# Autodesk Inventor assembly: Cold Plate in Box
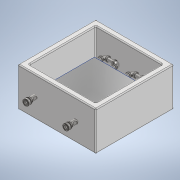
[picture p0: Inventor's stored thumbnail of the model, 180x180]
Saved by Autodesk Inventor 2022 (Build 260153000, 153)
## iProperties
Created: 2022-01-24
Part Number: Cold Plate in Box
Document SubType Name: Assembly
Designer: Caleb
Author: Caleb
## Documents named in this file (3)
- C:\Users\Caleb\Desktop\nebraska-silicon-lab\Hardware\TFPX\Cold Plate\Cold Plate in Box.iam
- C:\Users\Caleb\Desktop\nebraska-silicon-lab\Hardware\TFPX\Cold Plate\Cold Plate.iam
- C:\Users\Caleb\Desktop\nebraska-silicon-lab\Hardware\TFPX\Cold Plate\S-12685 Insulated Box.ipt
## Components (2 placed, 2 different names)
1. Cold Plate:1 [sub-assembly] — Angle:1, Angle:2
2. S-12685 Insulated Box:1 — Angle:1, Angle:2
## Relationships (2: Angle 2)
- Angle:1 (0 deg): Cold Plate:1 ↔ S-12685 Insulated Box:1
- Angle:2 (0 deg): Cold Plate:1 ↔ S-12685 Insulated Box:1
